# Autodesk Inventor assembly: MechSwitch_Assem_V3
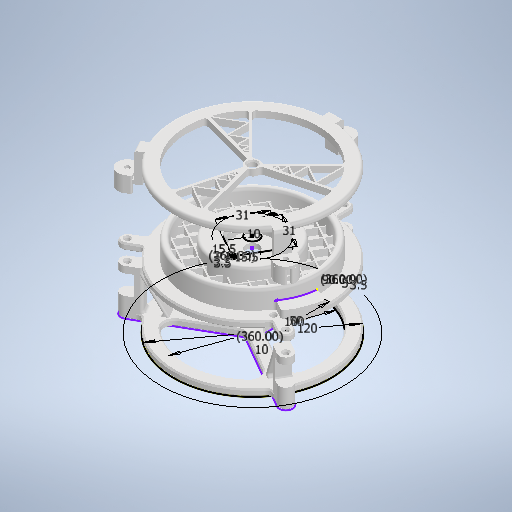
[picture p0: Inventor's stored thumbnail of the model, 512x512]
Saved by Autodesk Inventor 2025.1 (Build 291241000, 241)
## iProperties
Created: 2026-04-16
Part Number: MechSwitch_Assem_V3
Document SubType Name: Assembly
Designer: ryand
Author: ryand
## Documents named in this file (5)
- C:\Users\ryand\OneDrive\Documents\Inventor\TNG\Rotational_TENG\MechSwitch\MechSwitch_Assem_V3.iam
- C:\Users\ryand\OneDrive\Documents\Inventor\TNG\Rotational_TENG\MechSwitch\MechSwitch_MotorBaseiptV3.ipt
- C:\Users\ryand\OneDrive\Documents\Inventor\TNG\Rotational_TENG\MechSwitch\Bottom_Stand.ipt
- C:\Users\ryand\OneDrive\Documents\Inventor\TNG\Rotational_TENG\MechSwitch\MechSwitch_DielecTopV3.ipt
- C:\Users\ryand\OneDrive\Documents\Inventor\TNG\Rotational_TENG\MechSwitch\Align_Bracket.ipt
## Components (6 placed, 4 different names)
1. MechSwitch_MotorBaseiptV3:1 — Insert:1, Insert:2
2. Bottom_Stand:1 — Insert:1
3. MechSwitch_DielecTopV3:1 — Insert:2, Insert:3, Mate:1, Insert:4, Mate:2, Insert:5, Mate:3
4. Align_Bracket:1 — Insert:5, Mate:3
5. Align_Bracket:2 — Insert:4, Mate:2
6. Align_Bracket:3 — Insert:3, Mate:1
## Relationships (8: Insert 5, Mate 3)
- Insert:1 (10 mm): MechSwitch_MotorBaseiptV3:1 ↔ Bottom_Stand:1
- Insert:2 (40 mm): MechSwitch_MotorBaseiptV3:1 ↔ MechSwitch_DielecTopV3:1
- Insert:3 (2 mm): MechSwitch_DielecTopV3:1 ↔ Align_Bracket:3
- Mate:1 (0.5 mm): MechSwitch_DielecTopV3:1 ↔ Align_Bracket:3
- Insert:4 (2 mm): MechSwitch_DielecTopV3:1 ↔ Align_Bracket:2
- Mate:2 (0.5 mm): MechSwitch_DielecTopV3:1 ↔ Align_Bracket:2
- Insert:5 (2 mm): MechSwitch_DielecTopV3:1 ↔ Align_Bracket:1
- Mate:3 (0.5 mm): MechSwitch_DielecTopV3:1 ↔ Align_Bracket:1
